# Autodesk Inventor assembly: Universal Coupler 6mm
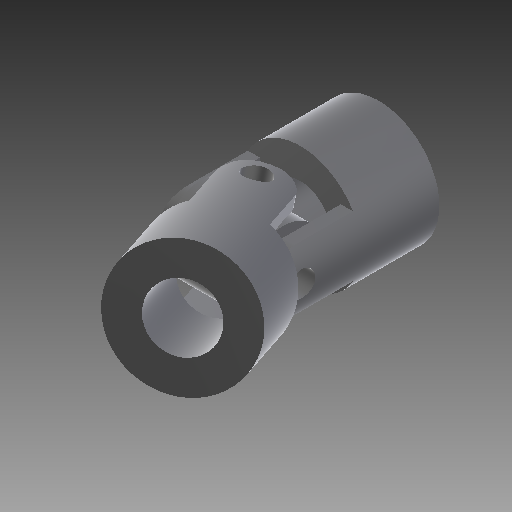
[picture p0: Inventor's stored thumbnail of the model, 512x512]
Saved by Autodesk Inventor 2017 SP1 (Build 210196100, 196)
## iProperties
Created: 2018-03-20
Part Number: Universal Coupler 6mm
Document SubType Name: Assembly
Designer: Zach
Author: Zach
## Documents named in this file (3)
- C:\Users\Zach\Documents\GitHub\tr1\lib\Universal Coupler, 6mm\Universal Coupler 6mm.iam
- C:\Users\Zach\Documents\GitHub\tr1\lib\Universal Coupler, 6mm\P1.ipt
- C:\Users\Zach\Documents\GitHub\tr1\lib\Universal Coupler, 6mm\P2.ipt
## Components (3 placed, 2 different names)
1. P1:1 — Mate:1, Mate:2
2. P2:1 — Mate:1, Mate:2, Mate:3, Tangent:1
3. P1:2 — Mate:3, Tangent:1
## Relationships (4: Mate 3, Tangent 1)
- Mate:1: P1:1 ↔ P2:1
- Mate:2: P1:1 ↔ P2:1
- Mate:3: P2:1 ↔ P1:2
- Tangent:1: P2:1 ↔ P1:2
